# Autodesk Inventor assembly: StandardPillarCover
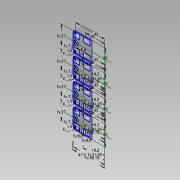
[picture p0: Inventor's stored thumbnail of the model, 180x180]
Saved by Autodesk Inventor 2021 (Build 250183000, 183)
## iProperties
Created: 2021-03-17
Part Number: StandardPillarCover
Document SubType Name: Assembly
Designer: kumagai
Author: kumagai
## Documents named in this file (2)
- X:\Develop\CAD\PlaRails\ViaductPillar\StandardPillarCover.iam
- X:\Develop\CAD\PlaRails\ViaductPillar\StandardPillarCover.ipt
## Components (4 placed, 1 different names)
1. StandardPillarCover:1
2. StandardPillarCover:2
3. StandardPillarCover:3
4. StandardPillarCover:4
## Component patterns: (4 elements, first: StandardPillarCover:1)
